# Autodesk Inventor assembly: SM-FA01
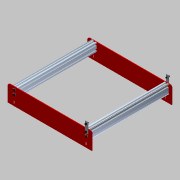
[picture p0: Inventor's stored thumbnail of the model, 180x180]
Saved by Autodesk Inventor 2012 SP1 (Build 160190100, 190)
## iProperties
Created: 2012-01-16
Part Number: SM-FA01
Document SubType Name: Assembly
Designer: ERF
Mass: 2459.09 g
Surface Area: 4000.62 cm^2
Volume: 486.549 cm^3
Density: 5.05415 g/cm^3
Author: ERF
Title: Shapeoko - Frame Assembly
## Documents named in this file (7)
- C:\Users\eford\Documents\Projects\Shapoko_v1i\Workspaces\Workspace\Projects\USER FOLDER\Edward\Shapeoko_v1i\Assemblies\SM-FA01.iam
- C:\Users\eford\Documents\Projects\Shapoko_v1i\Workspaces\Workspace\Projects\USER FOLDER\Edward\Shapeoko_v1i\Parts\SM-S02.ipt
- C:\Users\eford\Documents\Projects\Shapoko_v1i\Workspaces\Workspace\Projects\USER FOLDER\Edward\Shapeoko_v1i\Parts\SM-H03.ipt
- C:\Users\eford\Documents\Projects\Shapoko_v1i\Workspaces\Workspace\Projects\USER FOLDER\Edward\Shapeoko_v1i\Parts\SM-M05.ipt
- C:\Users\eford\Documents\Projects\Shapoko_v1i\Workspaces\Workspace\Projects\USER FOLDER\Edward\Shapeoko_v1i\Parts\SM-H11.ipt
- C:\Users\eford\Documents\Projects\Shapoko_v1i\Workspaces\Workspace\Projects\USER FOLDER\Edward\Shapeoko_v1i\Parts\SM-H07.ipt
- C:\Users\eford\Documents\Projects\Shapoko_v1i\Workspaces\Workspace\Projects\USER FOLDER\Edward\Shapeoko_v1i\Parts\MSK01-02.ipt
## Components (28 placed, 6 different names)
1. MSK01-02:2 — Insert:1, Insert:2, Insert:5, Insert:6
2. MSK01-02:1 — Insert:3, Insert:4, Insert:7, Insert:8
3. SM-S02:1 — Insert:1, Insert:2, Insert:3, Insert:4, Insert:14, Insert:25, Angle:1, Insert:29, Insert:31
4. SM-S02:2 — Insert:5, Insert:6, Insert:7, Insert:8, Insert:20, Insert:23, Insert:24, Insert:32, Angle:2
5. SM-H07:1 — Insert:10
6. SM-H07:2 — Insert:49
7. SM-H07:3 — Insert:47
8. SM-H07:4 — Insert:48
9. SM-H03:3 — Insert:24, Insert:47
10. SM-H03:4 — Insert:23, Insert:48
11. SM-H03:6 — Insert:10, Insert:14
12. SM-H03:7 — Insert:20, Insert:49
13. SM-M05:1 — Insert:25, Angle:1, Insert:26, Insert:36, Insert:42
14. SM-H07:5 — Insert:43
15. SM-H03:9 — Insert:26, Insert:43
16. SM-H07:6 — Insert:46
17. SM-H03:10 — Insert:29, Insert:46
18. SM-H07:7 — Insert:45
19. SM-H03:11 — Insert:31, Insert:45
20. SM-M05:2 — Insert:32, Angle:2, Insert:33, Insert:38, Insert:41
21. SM-H07:8 — Insert:50
22. SM-H03:12 — Insert:33, Insert:50
23. SM-H03:13 — Insert:36, Insert:44
24. SM-H07:9 — Insert:44
25. SM-H03:14 — Insert:38, Insert:51
26. SM-H07:10 — Insert:51
27. SM-H11:1 — Insert:41
28. SM-H11:2 — Insert:42
## Relationships (34: Insert 32, Angle 2)
- Insert:1: MSK01-02:2 ↔ SM-S02:1
- Insert:2: MSK01-02:2 ↔ SM-S02:1
- Insert:3: MSK01-02:1 ↔ SM-S02:1
- Insert:4: MSK01-02:1 ↔ SM-S02:1
- Insert:5: MSK01-02:2 ↔ SM-S02:2
- Insert:6: MSK01-02:2 ↔ SM-S02:2
- Insert:7: MSK01-02:1 ↔ SM-S02:2
- Insert:8: MSK01-02:1 ↔ SM-S02:2
- Insert:10: SM-H07:1 ↔ SM-H03:6
- Insert:14: SM-S02:1 ↔ SM-H03:6
- Insert:20: SM-S02:2 ↔ SM-H03:7
- Insert:23: SM-S02:2 ↔ SM-H03:4
- Insert:24: SM-S02:2 ↔ SM-H03:3
- Insert:25: SM-S02:1 ↔ SM-M05:1
- Angle:1 (0 deg): SM-S02:1 ↔ SM-M05:1
- Insert:26: SM-M05:1 ↔ SM-H03:9
- Insert:29: SM-S02:1 ↔ SM-H03:10
- Insert:31: SM-S02:1 ↔ SM-H03:11
- Insert:32: SM-S02:2 ↔ SM-M05:2
- Angle:2 (0 deg): SM-S02:2 ↔ SM-M05:2
- Insert:33: SM-M05:2 ↔ SM-H03:12
- Insert:36: SM-M05:1 ↔ SM-H03:13
- Insert:38: SM-M05:2 ↔ SM-H03:14
- Insert:41: SM-M05:2 ↔ SM-H11:1
- Insert:42: SM-M05:1 ↔ SM-H11:2
- Insert:43: SM-H07:5 ↔ SM-H03:9
- Insert:44: SM-H03:13 ↔ SM-H07:9
- Insert:45: SM-H07:7 ↔ SM-H03:11
- Insert:46: SM-H07:6 ↔ SM-H03:10
- Insert:47: SM-H07:3 ↔ SM-H03:3
- Insert:48: SM-H07:4 ↔ SM-H03:4
- Insert:49: SM-H07:2 ↔ SM-H03:7
- Insert:50: SM-H07:8 ↔ SM-H03:12
- Insert:51: SM-H03:14 ↔ SM-H07:10
